# Autodesk Inventor assembly: IntakeCCenterWheelPolyPlates
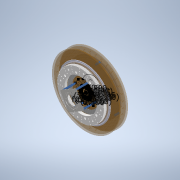
[picture p0: Inventor's stored thumbnail of the model, 180x180]
Saved by Autodesk Inventor 2020 (Build 240168000, 168)
## iProperties
Created: 2020-01-19
Part Number: IntakeCCenterWheelPolyPlates
Document SubType Name: Assembly
Designer: srini
Author: srini
## Documents named in this file (12)
- C:\Users\srini\Documents\FRC\2020\IntakeShooter\IntakeCCenterWheelPolyPlates.iam
- C:\Users\srini\Documents\FRC\2020\IntakeShooter\IndexerPolyWheelPlateSet.iam
- C:\Users\srini\Documents\FRC\2020\IntakeShooter\IndexWheelFlatPlatesPolyInside.ipt
- C:\Users\srini\Documents\FRC\2020\IntakeShooter\IndexWheelFlatPlatesPolyOutside.ipt
- C:\Users\srini\Documents\FRC\2020\FRC 2020 FIRSTChoice Inventor\Inventor\12C9045G.ipt
- C:\Users\srini\Documents\FRC\2020\IntakeShooter\Spacer3_8x1.ipt
- C:\Users\srini\Documents\FRC\2020\IntakeShooter\IntakeCCenterWheelInterposer.ipt
- C:\Users\srini\Documents\FRC\2020\IntakeShooter\152ToothBase.ipt
- C:\Users\srini\Documents\FRC\2020\IntakeShooter\Spacer3_8x2.ipt
- C:\Users\srini\Documents\FRC\2020\IntakeShooter\100ToothBase.ipt
- C:\Users\srini\Documents\FRC\2020\IntakeShooter\Spacer3_8x1.27.ipt
- C:\Users\srini\Documents\FRC\2020\FRC 2020 FIRSTChoice Inventor\Inventor\4C8135.iam
## Components (40 placed, 11 different names)
1. IndexerPolyWheelPlateSet:1 [sub-assembly] — Insert:1, Insert:2, Insert:7, Insert:8, Insert:9, Insert:10, Insert:11, Insert:12, Insert:34, Insert:35, Insert:36, Insert:37, Insert:38, Insert:39, Insert:40, Insert:41, Insert:42, Insert:43, Insert:44, Insert:45, Insert:46, Insert:47
2. IndexWheelFlatPlatesPolyInside:1 — Insert:1, Insert:2, Insert:3, Insert:4
3. IndexWheelFlatPlatesPolyOutside:1 — Insert:3, Insert:4, Insert:5, Insert:6, Insert:29, Insert:30, Insert:31, Insert:32
4. 12C9045G:1 — Insert:5, Insert:6, Mate:1, Mate:2
5. 12C9045G:2 — Insert:7, Insert:8, Mate:3, Mate:4
6. Spacer3_8x1:1 — Insert:9
7. Spacer3_8x1:2 — Insert:10
8. Spacer3_8x1:3 — Insert:11
9. Spacer3_8x1:4 — Insert:12
10. IntakeCCenterWheelInterposer:1 — Mate:1, Mate:2, Mate:5, Insert:13, Insert:14, Insert:15, Insert:16, Insert:17, Insert:18, Insert:19, Insert:20
11. IntakeCCenterWheelInterposer:2 — Mate:3, Mate:4, Mate:5, Insert:21, Insert:22, Insert:23, Insert:24, Insert:25, Insert:26, Insert:27, Insert:28
12. 152ToothBase:1 — Insert:19, Insert:20
13. 152ToothBase:2 — Insert:13, Insert:14
14. 152ToothBase:3 — Insert:15, Insert:16
15. 152ToothBase:4 — Insert:17, Insert:18
16. 152ToothBase:5 — Insert:21, Insert:22
17. 152ToothBase:6 — Insert:23, Insert:24
18. 152ToothBase:7 — Insert:25, Insert:26
19. 152ToothBase:8 — Insert:27, Insert:28
20. Spacer3_8x2:1 — Insert:31, Tangent:1
21. Spacer3_8x2:2 — Insert:37
22. Spacer3_8x2:3 — Insert:36, Mate:6, Insert:49
23. Spacer3_8x2:4 — Insert:32, Insert:48
24. Spacer3_8x2:5 — Insert:34, Tangent:2
25. Spacer3_8x2:7 — Insert:30
26. Spacer3_8x2:8 — Insert:29
27. Spacer3_8x2:9 — Insert:35
28. Spacer3_8x2:10 — Insert:39
29. Spacer3_8x2:11 — Insert:40
30. Spacer3_8x2:12 — Insert:38
31. Spacer3_8x2:13 — Insert:41
32. Spacer3_8x1.27:1 — Insert:45, Mate:8
33. Spacer3_8x1.27:2 — Insert:44
34. Spacer3_8x1.27:3 — Insert:47
35. Spacer3_8x1.27:4 — Insert:46
36. Spacer3_8x1.27:6 — Insert:43
37. Spacer3_8x1.27:8 — Insert:42, Mate:7
38. 100ToothBase:1 — Mate:6, Mate:7, Mate:8
39. 4C8135:1 [sub-assembly] — Insert:49, Tangent:2
40. 4C8135:2 [sub-assembly] — Insert:48, Tangent:1
## Relationships (58: Insert 48, Mate 8, Tangent 2)
- Insert:1 (25.4 mm): IndexerPolyWheelPlateSet:1 ↔ IndexWheelFlatPlatesPolyInside:1
- Insert:2 (25.4 mm): IndexerPolyWheelPlateSet:1 ↔ IndexWheelFlatPlatesPolyInside:1
- Insert:3: IndexWheelFlatPlatesPolyInside:1 ↔ IndexWheelFlatPlatesPolyOutside:1
- Insert:4: IndexWheelFlatPlatesPolyInside:1 ↔ IndexWheelFlatPlatesPolyOutside:1
- Insert:5: IndexWheelFlatPlatesPolyOutside:1 ↔ 12C9045G:1
- Insert:6: IndexWheelFlatPlatesPolyOutside:1 ↔ 12C9045G:1
- Insert:7: IndexerPolyWheelPlateSet:1 ↔ 12C9045G:2
- Insert:8: IndexerPolyWheelPlateSet:1 ↔ 12C9045G:2
- Insert:9: IndexerPolyWheelPlateSet:1 ↔ Spacer3_8x1:1
- Insert:10: IndexerPolyWheelPlateSet:1 ↔ Spacer3_8x1:2
- Insert:11: IndexerPolyWheelPlateSet:1 ↔ Spacer3_8x1:3
- Insert:12: IndexerPolyWheelPlateSet:1 ↔ Spacer3_8x1:4
- Mate:1: 12C9045G:1 ↔ IntakeCCenterWheelInterposer:1
- Mate:2: 12C9045G:1 ↔ IntakeCCenterWheelInterposer:1
- Mate:3: 12C9045G:2 ↔ IntakeCCenterWheelInterposer:2
- Mate:4: 12C9045G:2 ↔ IntakeCCenterWheelInterposer:2
- Mate:5: IntakeCCenterWheelInterposer:1 ↔ IntakeCCenterWheelInterposer:2
- Insert:13: IntakeCCenterWheelInterposer:1 ↔ 152ToothBase:2
- Insert:14: IntakeCCenterWheelInterposer:1 ↔ 152ToothBase:2
- Insert:15: IntakeCCenterWheelInterposer:1 ↔ 152ToothBase:3
- Insert:16: IntakeCCenterWheelInterposer:1 ↔ 152ToothBase:3
- Insert:17: IntakeCCenterWheelInterposer:1 ↔ 152ToothBase:4
- Insert:18: IntakeCCenterWheelInterposer:1 ↔ 152ToothBase:4
- Insert:19: IntakeCCenterWheelInterposer:1 ↔ 152ToothBase:1
- Insert:20: IntakeCCenterWheelInterposer:1 ↔ 152ToothBase:1
- Insert:21: IntakeCCenterWheelInterposer:2 ↔ 152ToothBase:5
- Insert:22: IntakeCCenterWheelInterposer:2 ↔ 152ToothBase:5
- Insert:23: IntakeCCenterWheelInterposer:2 ↔ 152ToothBase:6
- Insert:24: IntakeCCenterWheelInterposer:2 ↔ 152ToothBase:6
- Insert:25: IntakeCCenterWheelInterposer:2 ↔ 152ToothBase:7
- Insert:26: IntakeCCenterWheelInterposer:2 ↔ 152ToothBase:7
- Insert:27: IntakeCCenterWheelInterposer:2 ↔ 152ToothBase:8
- Insert:28: IntakeCCenterWheelInterposer:2 ↔ 152ToothBase:8
- Insert:29: IndexWheelFlatPlatesPolyOutside:1 ↔ Spacer3_8x2:8
- Insert:30: IndexWheelFlatPlatesPolyOutside:1 ↔ Spacer3_8x2:7
- Insert:31: IndexWheelFlatPlatesPolyOutside:1 ↔ Spacer3_8x2:1
- Insert:32: IndexWheelFlatPlatesPolyOutside:1 ↔ Spacer3_8x2:4
- Insert:34: IndexerPolyWheelPlateSet:1 ↔ Spacer3_8x2:5
- Insert:35: IndexerPolyWheelPlateSet:1 ↔ Spacer3_8x2:9
- Insert:36: IndexerPolyWheelPlateSet:1 ↔ Spacer3_8x2:3
- Insert:37: IndexerPolyWheelPlateSet:1 ↔ Spacer3_8x2:2
- Insert:38: IndexerPolyWheelPlateSet:1 ↔ Spacer3_8x2:12
- Insert:39: IndexerPolyWheelPlateSet:1 ↔ Spacer3_8x2:10
- Insert:40: IndexerPolyWheelPlateSet:1 ↔ Spacer3_8x2:11
- Insert:41: IndexerPolyWheelPlateSet:1 ↔ Spacer3_8x2:13
- Insert:42: IndexerPolyWheelPlateSet:1 ↔ Spacer3_8x1.27:8
- Insert:43: IndexerPolyWheelPlateSet:1 ↔ Spacer3_8x1.27:6
- Insert:44: IndexerPolyWheelPlateSet:1 ↔ Spacer3_8x1.27:2
- Insert:45: IndexerPolyWheelPlateSet:1 ↔ Spacer3_8x1.27:1
- Insert:46: IndexerPolyWheelPlateSet:1 ↔ Spacer3_8x1.27:4
- Insert:47: IndexerPolyWheelPlateSet:1 ↔ Spacer3_8x1.27:3
- Mate:6: Spacer3_8x2:3 ↔ 100ToothBase:1
- Mate:7: Spacer3_8x1.27:8 ↔ 100ToothBase:1
- Insert:48: Spacer3_8x2:4 ↔ 4C8135:2
- Tangent:1: Spacer3_8x2:1 ↔ 4C8135:2
- Insert:49: Spacer3_8x2:3 ↔ 4C8135:1
- Tangent:2: Spacer3_8x2:5 ↔ 4C8135:1
- Mate:8: Spacer3_8x1.27:1 ↔ 100ToothBase:1
